# Autodesk Inventor assembly: feet_fin1
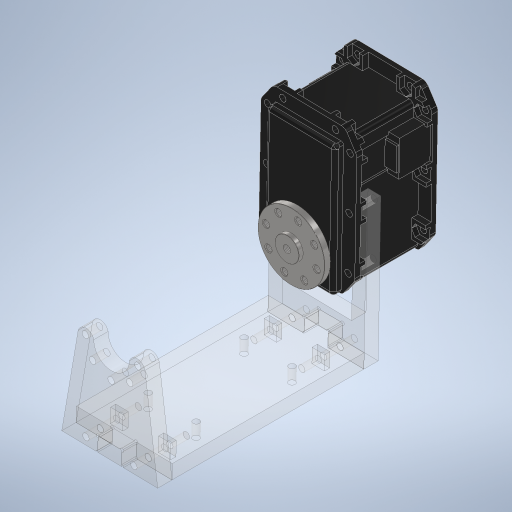
[picture p0: Inventor's stored thumbnail of the model, 512x512]
Saved by Autodesk Inventor 2024 (Build 280153000, 153)
## iProperties
Created: 2024-09-14
Part Number: feet_fin1
Document SubType Name: Assembly
Designer: jmha0
Author: jmha0
## Documents named in this file (6)
- C:\Users\jmha0\OneDrive\바탕 화면\19th_intern_hjm_fight_robot\Lower_Body\feet\feet_fin1.iam
- C:\Users\jmha0\OneDrive\바탕 화면\19th_intern_hjm_fight_robot\Lower_Body\feet\feet_holder3.ipt
- C:\Users\jmha0\OneDrive\바탕 화면\19th_intern_hjm_fight_robot\Lower_Body\feet\feet_holder1.ipt
- C:\Users\jmha0\OneDrive\바탕 화면\19th_intern_hjm_fight_robot\Lower_Body\feet\feet_holder2.ipt
- C:\Users\jmha0\OneDrive\바탕 화면\19th_intern_hjm_fight_robot\hardware\ROBOTIS(Inventor 2024 ver.)\다이나믹셀\MX-64T.ipt
- C:\Users\jmha0\OneDrive\바탕 화면\19th_intern_hjm_fight_robot\hardware\ROBOTIS(Inventor 2024 ver.)\혼\64-106Horn.ipt
## Components (5 placed, 5 different names)
1. feet_holder3:1 — 삽입:1, 삽입:2, 삽입:3, 삽입:4
2. feet_holder1:1 — 삽입:1, 삽입:2
3. feet_holder2:1 — 삽입:3, 삽입:4, 삽입:6, 삽입:7, 삽입:8, 삽입:9
4. MX-64T:1 — 삽입:5, 삽입:6, 삽입:7, 삽입:8, 삽입:9
5. 64-106Horn:1 — 삽입:5
## Relationships (9: Insert 9)
- 삽입:1 [Insert]: feet_holder3:1 ↔ feet_holder1:1
- 삽입:2 [Insert]: feet_holder3:1 ↔ feet_holder1:1
- 삽입:3 [Insert]: feet_holder3:1 ↔ feet_holder2:1
- 삽입:4 [Insert]: feet_holder3:1 ↔ feet_holder2:1
- 삽입:5 [Insert] (0.1 mm): MX-64T:1 ↔ 64-106Horn:1
- 삽입:6 [Insert] (2 mm): feet_holder2:1 ↔ MX-64T:1
- 삽입:7 [Insert] (2 mm): feet_holder2:1 ↔ MX-64T:1
- 삽입:8 [Insert] (2 mm): feet_holder2:1 ↔ MX-64T:1
- 삽입:9 [Insert] (2 mm): feet_holder2:1 ↔ MX-64T:1
